# Autodesk Inventor assembly: CAM_Assembly
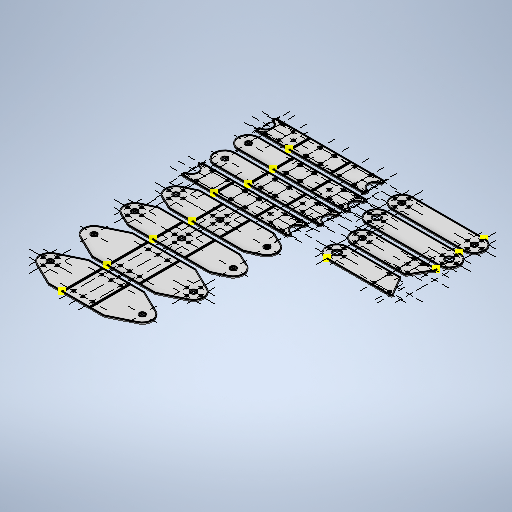
[picture p0: Inventor's stored thumbnail of the model, 512x512]
Saved by Autodesk Inventor 2025.2 (Build 292293000, 293)
## iProperties
Created: 2025-08-09
Part Number: CAM_Assembly
Document SubType Name: Assembly
Designer: User
Author: User
## Documents named in this file (13)
- C:\Users\User\Documents\The Maverick's Files\College 3-3\로보인 프로젝트\RHp_Humanoid_ver1\Part\Frame\Leg\Left Leg\CAM\CAM_Assembly.iam
- C:\Users\User\Documents\The Maverick's Files\College 3-3\로보인 프로젝트\RHp_Humanoid_ver1\Part\Frame\Leg\Left Leg\CAM\CAM_axis_1_top_frame.ipt
- C:\Users\User\Documents\The Maverick's Files\College 3-3\로보인 프로젝트\RHp_Humanoid_ver1\Part\Frame\Leg\Left Leg\CAM\CAM_axis_1_supplement_frame.ipt
- C:\Users\User\Documents\The Maverick's Files\College 3-3\로보인 프로젝트\RHp_Humanoid_ver1\Part\Frame\Leg\Left Leg\CAM\CAM_axis_2_4_connector_frame_non_powered.ipt
- C:\Users\User\Documents\The Maverick's Files\College 3-3\로보인 프로젝트\RHp_Humanoid_ver1\Part\Frame\Leg\Left Leg\CAM\CAM_axis_2_4_connector_frame_powered.ipt
- C:\Users\User\Documents\The Maverick's Files\College 3-3\로보인 프로젝트\RHp_Humanoid_ver1\Part\Frame\Leg\Left Leg\CAM\CAM_axis_2_bottom_frame.ipt
- C:\Users\User\Documents\The Maverick's Files\College 3-3\로보인 프로젝트\RHp_Humanoid_ver1\Part\Frame\Leg\Left Leg\CAM\CAM_axis_3_bottom_frame.ipt
- C:\Users\User\Documents\The Maverick's Files\College 3-3\로보인 프로젝트\RHp_Humanoid_ver1\Part\Frame\Leg\Left Leg\CAM\CAM_axis_4_5_connector_frame_non_powered.ipt
- C:\Users\User\Documents\The Maverick's Files\College 3-3\로보인 프로젝트\RHp_Humanoid_ver1\Part\Frame\Leg\Left Leg\CAM\CAM_axis_4_5_connector_frame_powered.ipt
- C:\Users\User\Documents\The Maverick's Files\College 3-3\로보인 프로젝트\RHp_Humanoid_ver1\Part\Frame\Leg\Left Leg\CAM\CAM_axis_5_top_frame.ipt
- C:\Users\User\Documents\The Maverick's Files\College 3-3\로보인 프로젝트\RHp_Humanoid_ver1\Part\Frame\Leg\Left Leg\CAM\CAM_axis_6_bottom_frame(top).ipt
- C:\Users\User\Documents\The Maverick's Files\College 3-3\로보인 프로젝트\RHp_Humanoid_ver1\Part\Frame\Leg\Left Leg\CAM\CAM_axis_6_supplement_frame.ipt
- C:\Users\User\Documents\The Maverick's Files\College 3-3\로보인 프로젝트\RHp_Humanoid_ver1\Part\Frame\Leg\Left Leg\CAM\CAM_axis_6_top_frame.ipt
## Components (12 placed, 12 different names)
1. CAM_axis_1_top_frame:1 — Flush:1, Flush:2, Flush:3, Mate:1, Flush:4, Flush:5, Flush:6, Mate:4, Flush:7, Flush:8, Flush:9, Flush:10, Flush:11, Mate:7, Mate:8, Mate:6
2. CAM_axis_1_supplement_frame:1 — Mate:1, Mate:2, Flush:4, Mate:4, Mate:5
3. CAM_axis_2_4_connector_frame_non_powered:1 — Flush:16, Mate:17, Mate:21
4. CAM_axis_2_4_connector_frame_powered:1 — Flush:7, Flush:15, Flush:16, Mate:16, Mate:17, Mate:19
5. CAM_axis_2_bottom_frame:1 — Mate:2, Mate:3, Flush:5, Mate:5, Mate:14, Mate:21
6. CAM_axis_3_bottom_frame:1 — Mate:3, Flush:6, Mate:6, Mate:11, Mate:12, Mate:19
7. CAM_axis_4_5_connector_frame_non_powered:1 — Flush:14, Flush:15, Mate:15, Mate:16, Mate:20
8. CAM_axis_4_5_connector_frame_powered:1 — Flush:12, Flush:13, Flush:14, Mate:15, Mate:18
9. CAM_axis_5_top_frame:1 — Flush:10, Mate:13, Mate:14, Flush:12, Flush:13, Mate:18
10. CAM_axis_6_bottom_frame(top):1 — Flush:9, Mate:7, Mate:8, Mate:9, Mate:10
11. CAM_axis_6_supplement_frame:1 — Flush:8, Mate:9, Mate:10
12. CAM_axis_6_top_frame:1 — Flush:11, Mate:11, Mate:12, Mate:13, Mate:20
## Relationships (37: Mate 21, Flush 16)
- Flush:1: CAM_axis_1_top_frame:1
- Flush:2: CAM_axis_1_top_frame:1
- Flush:3: CAM_axis_1_top_frame:1
- Mate:1 (5 mm): CAM_axis_1_top_frame:1 ↔ CAM_axis_1_supplement_frame:1
- Mate:2 (5 mm): CAM_axis_1_supplement_frame:1 ↔ CAM_axis_2_bottom_frame:1
- Mate:3 (5 mm): CAM_axis_2_bottom_frame:1 ↔ CAM_axis_3_bottom_frame:1
- Flush:4: CAM_axis_1_top_frame:1 ↔ CAM_axis_1_supplement_frame:1
- Flush:5: CAM_axis_1_top_frame:1 ↔ CAM_axis_2_bottom_frame:1
- Flush:6: CAM_axis_1_top_frame:1 ↔ CAM_axis_3_bottom_frame:1
- Mate:4: CAM_axis_1_top_frame:1 ↔ CAM_axis_1_supplement_frame:1
- Mate:5: CAM_axis_1_supplement_frame:1 ↔ CAM_axis_2_bottom_frame:1
- Mate:6: CAM_axis_1_top_frame:1 ↔ CAM_axis_3_bottom_frame:1
- Flush:7: CAM_axis_1_top_frame:1 ↔ CAM_axis_2_4_connector_frame_powered:1
- Flush:8: CAM_axis_1_top_frame:1 ↔ CAM_axis_6_supplement_frame:1
- Flush:9: CAM_axis_1_top_frame:1 ↔ CAM_axis_6_bottom_frame(top):1
- Flush:10: CAM_axis_1_top_frame:1 ↔ CAM_axis_5_top_frame:1
- Flush:11: CAM_axis_1_top_frame:1 ↔ CAM_axis_6_top_frame:1
- Mate:7 (5 mm): CAM_axis_1_top_frame:1 ↔ CAM_axis_6_bottom_frame(top):1
- Mate:8: CAM_axis_1_top_frame:1 ↔ CAM_axis_6_bottom_frame(top):1
- Mate:9 (5 mm): CAM_axis_6_bottom_frame(top):1 ↔ CAM_axis_6_supplement_frame:1
- Mate:10: CAM_axis_6_bottom_frame(top):1 ↔ CAM_axis_6_supplement_frame:1
- Mate:11 (5 mm): CAM_axis_3_bottom_frame:1 ↔ CAM_axis_6_top_frame:1
- Mate:12: CAM_axis_3_bottom_frame:1 ↔ CAM_axis_6_top_frame:1
- Mate:13 (5 mm): CAM_axis_5_top_frame:1 ↔ CAM_axis_6_top_frame:1
- Mate:14: CAM_axis_2_bottom_frame:1 ↔ CAM_axis_5_top_frame:1
- Flush:12: CAM_axis_4_5_connector_frame_powered:1 ↔ CAM_axis_5_top_frame:1
- Flush:13: CAM_axis_4_5_connector_frame_powered:1 ↔ CAM_axis_5_top_frame:1
- Flush:14: CAM_axis_4_5_connector_frame_non_powered:1 ↔ CAM_axis_4_5_connector_frame_powered:1
- Flush:15: CAM_axis_2_4_connector_frame_powered:1 ↔ CAM_axis_4_5_connector_frame_non_powered:1
- Flush:16: CAM_axis_2_4_connector_frame_non_powered:1 ↔ CAM_axis_2_4_connector_frame_powered:1
- Mate:15 (5 mm): CAM_axis_4_5_connector_frame_non_powered:1 ↔ CAM_axis_4_5_connector_frame_powered:1
- Mate:16 (5 mm): CAM_axis_2_4_connector_frame_powered:1 ↔ CAM_axis_4_5_connector_frame_non_powered:1
- Mate:17 (5 mm): CAM_axis_2_4_connector_frame_non_powered:1 ↔ CAM_axis_2_4_connector_frame_powered:1
- Mate:18 (20 mm): CAM_axis_4_5_connector_frame_powered:1 ↔ CAM_axis_5_top_frame:1
- Mate:19 (-25 mm): CAM_axis_2_4_connector_frame_powered:1 ↔ CAM_axis_3_bottom_frame:1
- Mate:20 (13 mm): CAM_axis_4_5_connector_frame_non_powered:1 ↔ CAM_axis_6_top_frame:1
- Mate:21 (32 mm): CAM_axis_2_4_connector_frame_non_powered:1 ↔ CAM_axis_2_bottom_frame:1
